# Autodesk Inventor assembly: korp
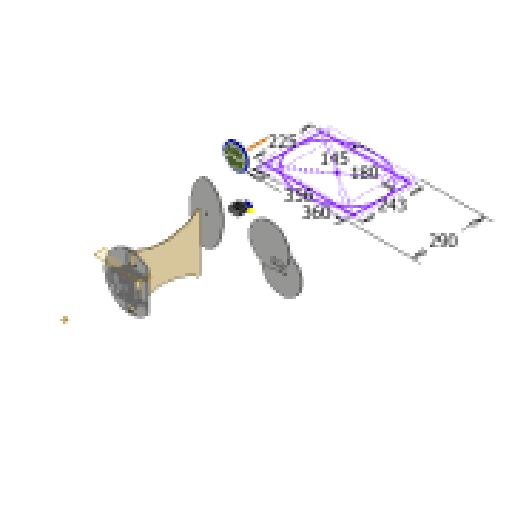
[picture p0: Inventor's stored thumbnail of the model, 512x512]
Saved by Autodesk Inventor 2023.2 (Build 272271030, 271C)
## iProperties
Created: 2023-03-13
Part Number: korp
Document SubType Name: Assembly
Designer: User
Author: User
## Documents named in this file (16)
- D:\!Cheburashka\Cheburashka\Cheburashka_construction\korpus\korp.iam
- D:\!Cheburashka\Cheburashka\Cheburashka_construction\korpus\нижний эллипс тела.ipt
- D:\!Cheburashka\Cheburashka\Cheburashka_construction\korpus\грань тела.ipt
- D:\!Cheburashka\Cheburashka\Cheburashka_construction\korpus\верхний эллипс туловища.ipt
- D:\!Cheburashka\Cheburashka\Cheburashka_construction\korpus\нижний эллипс головы.ipt
- D:\!Cheburashka\Cheburashka\Cheburashka_construction\korpus\Servo.ipt
- D:\!Cheburashka\Cheburashka\Cheburashka_construction\korpus\Pitsco Education-739028.ipt
- D:\!Cheburashka\Cheburashka\Cheburashka_construction\korpus\Pitsco Education-739085.ipt
- D:\!Cheburashka\Cheburashka\Cheburashka_construction\korpus\трубка.ipt
- D:\!Cheburashka\Cheburashka\Cheburashka_construction\korpus\Prostavka.ipt
- D:\!Cheburashka\Cheburashka\Cheburashka_construction\korpus\лицо1.ipt
- D:\!Cheburashka\Cheburashka\Cheburashka_construction\korpus\att_pin.ipt
- D:\!Cheburashka\Cheburashka\Cheburashka_construction\platform\print\Деталь1.ipt
- D:\!Cheburashka\Cheburashka\Cheburashka_construction\platform\KRAVT_holder_2 (1).ipt
- D:\!Cheburashka\Cheburashka\Cheburashka_construction\korpus\ребро.ipt
- D:\!Cheburashka\Cheburashka\Cheburashka_construction\korpus\ребро_MIR.ipt
## Components (16 placed, 15 different names)
1. нижний эллипс тела:1 — Совмещение:100, Симметрия:1
2. верхний эллипс туловища:1
3. грань тела:1 — Совмещение:101, Заподлицо:19
4. нижний эллипс головы:1 — Совмещение:73
5. Pitsco Education-739028:1 — Совмещение:99
6. Pitsco Education-739085:1 — Совмещение:68, Совмещение:75, Совмещение:80
7. трубка:1 — Совмещение:68, Совмещение:74, Совмещение:81
8. Servo:4 — Совмещение:97, Совмещение:98
9. Prostavka:1 — Совмещение:73, Совмещение:74, Совмещение:75
10. Prostavka:2 — Совмещение:80, Совмещение:81, Заподлицо:16
11. лицо1:1 — Заподлицо:16, Заподлицо:17
12. att_pin:1 — Совмещение:97, Совмещение:98, Совмещение:99
13. Деталь1:1 — Заподлицо:17
14. KRAVT_holder_2 (1):1 — Совмещение:100, Совмещение:101, Симметрия:1
15. ребро:1 — Заподлицо:18
16. ребро_MIR:1 — Совмещение:102
## Relationships (17: Mate 12, Flush 4, Symmetry 1)
- Совмещение:68 [Mate]: Pitsco Education-739085:1 ↔ трубка:1
- Совмещение:73 [Mate]: нижний эллипс головы:1 ↔ Prostavka:1
- Совмещение:74 [Mate]: трубка:1 ↔ Prostavka:1
- Совмещение:75 [Mate]: Pitsco Education-739085:1 ↔ Prostavka:1
- Совмещение:80 [Mate]: Pitsco Education-739085:1 ↔ Prostavka:2
- Совмещение:81 [Mate]: трубка:1 ↔ Prostavka:2
- Заподлицо:16 [Flush]: Prostavka:2 ↔ лицо1:1
- Совмещение:97 [Mate]: Servo:4 ↔ att_pin:1
- Совмещение:98 [Mate]: Servo:4 ↔ att_pin:1
- Совмещение:99 [Mate]: Pitsco Education-739028:1 ↔ att_pin:1
- Заподлицо:17 [Flush]: лицо1:1 ↔ Деталь1:1
- Совмещение:100 [Mate]: нижний эллипс тела:1 ↔ KRAVT_holder_2 (1):1
- Совмещение:101 [Mate] (56.5 mm): грань тела:1 ↔ KRAVT_holder_2 (1):1
- Симметрия:1 [Symmetry]: нижний эллипс тела:1 ↔ KRAVT_holder_2 (1):1
- Заподлицо:18 [Flush]: ребро:1
- Заподлицо:19 [Flush] (-22.5399 mm): грань тела:1
- Совмещение:102 [Mate]: ребро_MIR:1
